# Autodesk Inventor assembly: Ring Gear
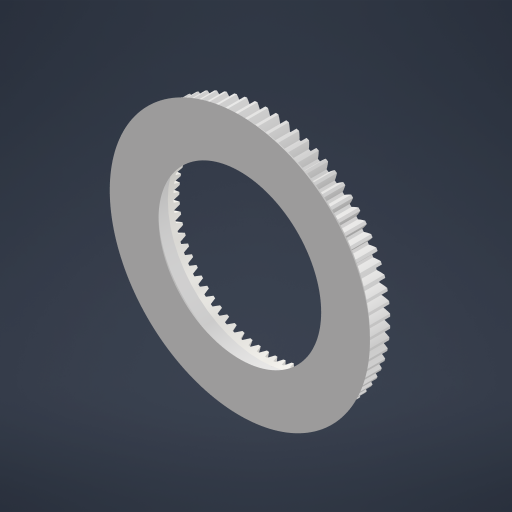
[picture p0: Inventor's stored thumbnail of the model, 512x512]
Saved by Autodesk Inventor 2023 (Build 270158000, 158)
## iProperties
Created: 2023-08-14
Part Number: Ring Gear
Document SubType Name: Assembly
Designer: Izack Waczko
Author: Izack Waczko
## Documents named in this file (4)
- F:\CAD Modeling\Private Robotics\Custom Tryhard Robot\Drivetrain\Custom-Modules-CAD\Differential Swerve Drive V1\Differential Swerve Drive Parts\Ring Gear.iam
- F:\CAD Modeling\Private Robotics\Custom Tryhard Robot\Drivetrain\Custom-Modules-CAD\Differential Swerve Drive V1\Ring Gear Base.ipt
- F:\CAD Modeling\Private Robotics\Custom Tryhard Robot\Drivetrain\Custom-Modules-CAD\Differential Swerve Drive V1\Differential Swerve Drive V1\Design Accelerator\Bevel Gear11.ipt
- F:\CAD Modeling\Private Robotics\Custom Tryhard Robot\Drivetrain\Custom-Modules-CAD\Differential Swerve Drive V1\Differential Swerve Drive Parts\OuterRing.ipt
## Components (3 placed, 3 different names)
1. Ring Gear Base:1 — Mate:1, Mate:2, Rigid:1, Flush:1, Flush:2
2. Bevel Gear1:1 — Mate:1, Mate:2, Rigid:1
3. OuterRing:1 — Flush:1, Flush:2
## Relationships (5: Mate 2, Flush 2, WeldJoint 1)
- Mate:1: Ring Gear Base:1 ↔ Bevel Gear1:1
- Mate:2: Ring Gear Base:1 ↔ Bevel Gear1:1
- Rigid:1 [WeldJoint]: Ring Gear Base:1 ↔ Bevel Gear1:1
- Flush:1: Ring Gear Base:1 ↔ OuterRing:1
- Flush:2: Ring Gear Base:1 ↔ OuterRing:1
